# Autodesk Inventor assembly: Rodamiento doble + arandela + cilindro separador
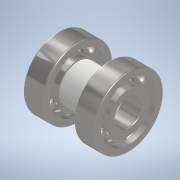
[picture p0: Inventor's stored thumbnail of the model, 180x180]
Saved by Autodesk Inventor 2021 (Build 250183000, 183)
## iProperties
Created: 2021-01-10
Part Number: Rodamiento doble + arandela + cilindro separador
Document SubType Name: Assembly
Designer: dieku
Author: dieku
## Documents named in this file (4)
- C:\Users\dieku\Documents\GitHub\tallerDibujoIngenieria\Ensambles\Rodamiento doble + arandela + cilindro separador.iam
- C:\Users\dieku\Documents\GitHub\tallerDibujoIngenieria\Ensambles\Rodamiento mas arandela.iam
- C:\Users\dieku\Documents\GitHub\tallerDibujoIngenieria\Partes\anilloseparador.ipt
- C:\Users\dieku\Documents\Inventor\Content Center Files\R2021\en-US\DIN 625 - T1\DIN 625 T1 - 6304 - 20 x 52 x 15.ipt
## Components (3 placed, 3 different names)
1. Rodamiento mas arandela:1 [sub-assembly] — Mate:1, Mate:2
2. anilloseparador:1 — Mate:1, Mate:2, Mate:3
3. DIN 625 - T1 6304 - 20 x 52 x 15:1 — Mate:3
## Relationships (3: Mate 3)
- Mate:1: Rodamiento mas arandela:1 ↔ anilloseparador:1
- Mate:2: Rodamiento mas arandela:1 ↔ anilloseparador:1
- Mate:3: anilloseparador:1 ↔ DIN 625 - T1 6304 - 20 x 52 x 15:1
